# Autodesk Inventor assembly: 3A.01.06.JS.Rib 6
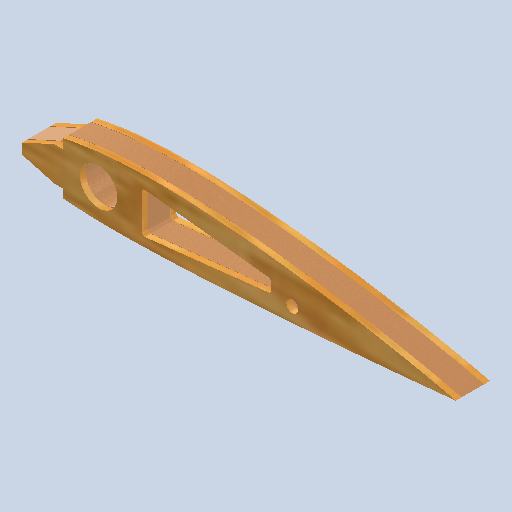
[picture p0: Inventor's stored thumbnail of the model, 512x512]
Saved by Autodesk Inventor 2025.1 (Build 291241000, 241)
## iProperties
Created: 2025-01-14
Part Number: 3A.01.06.JS.Rib 6
Document SubType Name: Assembly
Designer: johan
Author: johan
## Documents named in this file (3)
- C:\Users\johan\OneDrive - University of Bristol\CAD docs\2) Wing\2) Ribs\assemblies\3A.01.06.JS.Rib 6.iam
- C:\Users\johan\OneDrive - University of Bristol\CAD docs\2) Wing\2) Ribs\parts\Full length unmodified\3P.03.06.01.JS.rib 6 ply.ipt
- C:\Users\johan\OneDrive - University of Bristol\CAD docs\2) Wing\2) Ribs\parts\Full length unmodified\3P.03.06.02.JS.rib 6 foam.ipt
## Components (3 placed, 2 different names)
1. 3P.03.06.01.JS.rib 6 ply:1 — Rigid:1
2. 3P.03.06.02.JS.rib 6 foam:1 — Rigid:2, Rigid:1
3. 3P.03.06.01.JS.rib 6 ply:2 — Rigid:2
## Relationships (2: WeldJoint 2)
- Rigid:2 [WeldJoint]: 3P.03.06.02.JS.rib 6 foam:1 ↔ 3P.03.06.01.JS.rib 6 ply:2
- Rigid:1 [WeldJoint]: 3P.03.06.01.JS.rib 6 ply:1 ↔ 3P.03.06.02.JS.rib 6 foam:1
